# Autodesk Inventor assembly: ChainGuardAssembly
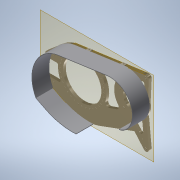
[picture p0: Inventor's stored thumbnail of the model, 180x180]
Saved by Autodesk Inventor 2021 (Build 250183000, 183)
## iProperties
Created: 2020-10-28
Part Number: ChainGuardAssembly
Document SubType Name: Assembly
Designer: PhotonUser
Quantity: 1
Author: PhotonUser
## Documents named in this file (3)
- D:\PhotonUser\Downloads\Assembly Files-20201028T000017Z-001\Assembly Files\ChainGuardAssembly.iam
- D:\PhotonUser\Downloads\Assembly Files-20201028T000017Z-001\Assembly Files\DiffMountRightipt.ipt
- D:\PhotonUser\Downloads\Assembly Files-20201028T000017Z-001\Assembly Files\ChainGuard.ipt
## Components (2 placed, 2 different names)
1. DiffMountRightipt:1 — Flush:1, Flush:2, Flush:3, Flush:6
2. ChainGuard:1 — Flush:1, Flush:2, Flush:3, Flush:6
## Relationships (4: Flush 4)
- Flush:1: DiffMountRightipt:1 ↔ ChainGuard:1
- Flush:2: DiffMountRightipt:1 ↔ ChainGuard:1
- Flush:3: DiffMountRightipt:1 ↔ ChainGuard:1
- Flush:6: DiffMountRightipt:1 ↔ ChainGuard:1
